# Autodesk Inventor assembly: Claw_1
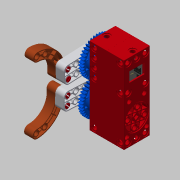
[picture p0: Inventor's stored thumbnail of the model, 180x180]
Saved by Autodesk Inventor 2019.3 (Build 233278000, 278)
## iProperties
Created: 2019-03-18
Part Number: Claw_1
Document SubType Name: Assembly
Designer: Varga Daniel
Author: Varga Daniel
## Documents named in this file (8)
- C:\!_Dani\!_cloud\OneDrive\!_munka\Revolution\RevvyDemoKit\Structural parts\Test assemblies\Claw_small_2.iam
- C:\!_Dani\!_cloud\OneDrive\!_munka\Revolution\RevvyDemoKit\Structural parts\Connetor Pins\CP1+x1+\CP1x1.ipt
- C:\!_Dani\!_cloud\OneDrive\!_munka\Revolution\RevvyDemoKit\Structural parts\Gears\G40.ipt
- C:\!_Dani\!_cloud\OneDrive\!_munka\Revolution\RevvyDemoKit\Structural parts\Demo parts\Motor\Inventor imported\motor.iam
- C:\!_Dani\!_cloud\OneDrive\!_munka\Revolution\RevvyDemoKit\Structural parts\Axles\AXp2p.ipt
- C:\!_Dani\!_cloud\OneDrive\!_munka\Revolution\RevvyDemoKit\Structural parts\Beams\Straight Beams\S2+x2\S4x2.ipt
- C:\!_Dani\!_cloud\OneDrive\!_munka\Revolution\RevvyDemoKit\Structural parts\Beams\Curved beams\CB4H.ipt
- C:\!_Dani\!_cloud\OneDrive\!_munka\Revolution\RevvyDemoKit\Structural parts\Connetor Pins\CP1+x1+\CP2x1.ipt
## Components (17 placed, 7 different names)
1. CB4H:1 — Insert:14, Insert:15
2. G40:1 — Mate:6, Angle:1, Insert:7, Rotation:1, Insert:20, Insert:21, Insert:23
3. motor:1 [sub-assembly] — Mate:1, Flush:1, Mate:2, Insert:5, Mate:6, Angle:2, Mate:7
4. AXp2p:1 — Mate:3, Mate:4, Mate:5, Insert:5
5. G40:2 — Mate:3, Mate:4, Mate:5, Angle:1, Angle:2, Rotation:1, Insert:24, Insert:25
6. CP1x1:3 — Insert:7, Mate:7
7. CB4H:2 — Insert:10, Insert:11
8. S4x2:1 — Insert:8, Insert:9, Insert:22, Insert:28
9. S4x2:2 — Insert:12, Insert:13, Insert:26, Insert:27
10. CP1x1:4 — Insert:8, Insert:10
11. CP1x1:5 — Insert:9, Insert:11
12. CP1x1:6 — Insert:12, Insert:14
13. CP1x1:7 — Insert:13, Insert:15
14. CP1x1:8 — Insert:25, Insert:27
15. CP1x1:9 — Insert:21, Insert:23, Insert:28
16. CP2x1:1 — Insert:20, Insert:22
17. CP1x1:10 — Insert:24, Insert:26
## Relationships (30: Insert 19, Mate 7, Angle 2, Flush 1, RelateRotation 1)
- Mate:1: motor:1
- Flush:1: motor:1
- Mate:2: motor:1
- Mate:3: AXp2p:1 ↔ G40:2
- Mate:4: AXp2p:1 ↔ G40:2
- Mate:5: AXp2p:1 ↔ G40:2
- Insert:5: motor:1 ↔ AXp2p:1
- Mate:6: G40:1 ↔ motor:1
- Angle:1 (0 deg): G40:1 ↔ G40:2
- Angle:2 (0 deg): motor:1 ↔ G40:2
- Insert:7: G40:1 ↔ CP1x1:3
- Mate:7: motor:1 ↔ CP1x1:3
- Insert:8: S4x2:1 ↔ CP1x1:4
- Insert:9: S4x2:1 ↔ CP1x1:5
- Insert:10: CB4H:2 ↔ CP1x1:4
- Insert:11: CB4H:2 ↔ CP1x1:5
- Insert:12: S4x2:2 ↔ CP1x1:6
- Insert:13: S4x2:2 ↔ CP1x1:7
- Insert:14: CB4H:1 ↔ CP1x1:6
- Insert:15: CB4H:1 ↔ CP1x1:7
- Rotation:1 [RelateRotation] (1 ul): G40:1 ↔ G40:2
- Insert:20: G40:1 ↔ CP2x1:1
- Insert:21: G40:1 ↔ CP1x1:9
- Insert:22: S4x2:1 ↔ CP2x1:1
- Insert:23: G40:1 ↔ CP1x1:9
- Insert:24: G40:2 ↔ CP1x1:10
- Insert:25: G40:2 ↔ CP1x1:8
- Insert:26: S4x2:2 ↔ CP1x1:10
- Insert:27: S4x2:2 ↔ CP1x1:8
- Insert:28: S4x2:1 ↔ CP1x1:9
